# Autodesk Inventor assembly: body assy
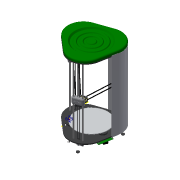
[picture p0: Inventor's stored thumbnail of the model, 180x180]
Saved by Autodesk Inventor 2016 (Build 200138000, 138)
## iProperties
Created: 2016-12-29
Part Number: body assy
Document SubType Name: Assembly
Designer: admin
Author: admin
## Documents named in this file (21)
- C:\Users\Juny\OneDrive - (주)에이팀벤처스\ateam\CL 3D프린터 사업- 설계 이준영\(((( delta 3D printer))))\20. 20190104 D3\1612 D3 3D modeling\body assy.iam
- C:\Users\Juny\OneDrive - (주)에이팀벤처스\ateam\CL 3D프린터 사업- 설계 이준영\(((( delta 3D printer))))\20. 20190104 D3\1612 D3 3D modeling\m3 6 socket_screw.ipt
- C:\Users\Juny\OneDrive - (주)에이팀벤처스\ateam\CL 3D프린터 사업- 설계 이준영\(((( delta 3D printer))))\20. 20190104 D3\1612 D3 3D modeling\m3 8 socket_screw.ipt
- C:\Users\Juny\OneDrive - (주)에이팀벤처스\ateam\CL 3D프린터 사업- 설계 이준영\(((( delta 3D printer))))\20. 20190104 D3\1612 D3 3D modeling\M3 16 BH_tapping_screw.ipt
- C:\Users\Juny\OneDrive - (주)에이팀벤처스\ateam\CL 3D프린터 사업- 설계 이준영\(((( delta 3D printer))))\20. 20190104 D3\1612 D3 3D modeling\m3 30 pcb_support.ipt
- C:\Users\Juny\OneDrive - (주)에이팀벤처스\ateam\CL 3D프린터 사업- 설계 이준영\(((( delta 3D printer))))\20. 20190104 D3\1612 D3 3D modeling\m4 10 Button Head.ipt
- C:\Users\Juny\OneDrive - (주)에이팀벤처스\ateam\CL 3D프린터 사업- 설계 이준영\(((( delta 3D printer))))\20. 20190104 D3\1612 D3 3D modeling\m4 12 Button Head.ipt
- C:\Users\Juny\OneDrive - (주)에이팀벤처스\ateam\CL 3D프린터 사업- 설계 이준영\(((( delta 3D printer))))\20. 20190104 D3\1612 D3 3D modeling\m4 20 Button Head.ipt
- C:\Users\Juny\OneDrive - (주)에이팀벤처스\ateam\CL 3D프린터 사업- 설계 이준영\(((( delta 3D printer))))\20. 20190104 D3\1612 D3 3D modeling\main_board.ipt
- C:\Users\Juny\OneDrive - (주)에이팀벤처스\ateam\CL 3D프린터 사업- 설계 이준영\(((( delta 3D printer))))\20. 20190104 D3\1612 D3 3D modeling\post.ipt
- C:\Users\Juny\OneDrive - (주)에이팀벤처스\ateam\CL 3D프린터 사업- 설계 이준영\(((( delta 3D printer))))\20. 20190104 D3\1612 D3 3D modeling\timing_belt.ipt
- C:\Users\Juny\OneDrive - (주)에이팀벤처스\ateam\CL 3D프린터 사업- 설계 이준영\(((( delta 3D printer))))\20. 20190104 D3\1612 D3 3D modeling\top_cover.ipt
- C:\Users\Juny\OneDrive - (주)에이팀벤처스\ateam\CL 3D프린터 사업- 설계 이준영\(((( delta 3D printer))))\20. 20190104 D3\1612 D3 3D modeling\back_cover.ipt
- C:\Users\Juny\OneDrive - (주)에이팀벤처스\ateam\CL 3D프린터 사업- 설계 이준영\(((( delta 3D printer))))\20. 20190104 D3\1612 D3 3D modeling\bottom cover assy\bottom cover assy.iam
- C:\Users\Juny\OneDrive - (주)에이팀벤처스\ateam\CL 3D프린터 사업- 설계 이준영\(((( delta 3D printer))))\20. 20190104 D3\1612 D3 3D modeling\bottom plate assy\bottom plate assy.iam
- C:\Users\Juny\OneDrive - (주)에이팀벤처스\ateam\CL 3D프린터 사업- 설계 이준영\(((( delta 3D printer))))\20. 20190104 D3\1612 D3 3D modeling\head assy\head assy.iam
- C:\Users\Juny\OneDrive - (주)에이팀벤처스\ateam\CL 3D프린터 사업- 설계 이준영\(((( delta 3D printer))))\20. 20190104 D3\1612 D3 3D modeling\lift block assy\lift block assy.iam
- C:\Users\Juny\OneDrive - (주)에이팀벤처스\ateam\CL 3D프린터 사업- 설계 이준영\(((( delta 3D printer))))\20. 20190104 D3\1612 D3 3D modeling\lod assy\lod assy.iam
- C:\Users\Juny\OneDrive - (주)에이팀벤처스\ateam\CL 3D프린터 사업- 설계 이준영\(((( delta 3D printer))))\20. 20190104 D3\1612 D3 3D modeling\motor assy\motor assy.iam
- C:\Users\Juny\OneDrive - (주)에이팀벤처스\ateam\CL 3D프린터 사업- 설계 이준영\(((( delta 3D printer))))\20. 20190104 D3\1612 D3 3D modeling\oled assy\oled assy.iam
- C:\Users\Juny\OneDrive - (주)에이팀벤처스\ateam\CL 3D프린터 사업- 설계 이준영\(((( delta 3D printer))))\20. 20190104 D3\1612 D3 3D modeling\top plate assy\top plate assy.iam
## Components (64 placed, 20 different names)
1. m3 6 socket_screw:1 — Rotational:39
2. M3 16 BH_tapping_screw:1 — Rotational:18
3. m3 30 pcb_support:1 — Rotational:33
4. m4 10 Button Head:1 — Rotational:25
5. m4 12 Button Head:1 — Rotational:32
6. main_board:1 — Rotational:37, Rotational:38, Rotational:39, Rotational:40, Rotational:41, Rotational:42
7. top_cover:1 — Rotational:23, Rotational:24
8. back_cover:1 — Rotational:21, Rotational:22, Rotational:25, Rotational:26, Rotational:27, Rotational:28, Rotational:29, Rotational:30, Rotational:31, Rotational:32
9. bottom cover assy:1 [sub-assembly] — Rotational:43, Rotational:44
10. bottom plate assy:1 [sub-assembly] — Rotational:3, Rotational:4, Rotational:5, Rotational:6, Rotational:7, Rotational:8, Rotational:21, Rotational:22, Angle:1, Angle:3, Angle:4, Rotational:33, Rotational:34, Rotational:35, Rotational:36, Rotational:43, Rotational:44
11. head assy:1 [sub-assembly] — Tangent:7, Tangent:8, Tangent:9, Tangent:10, Tangent:11, Tangent:12
12. lod assy:1 [sub-assembly] — Tangent:1, Tangent:8
13. oled assy:1 [sub-assembly] — Rotational:5, Rotational:6, Rotational:14, Rotational:15, Rotational:16, Rotational:17
14. top plate assy:1 [sub-assembly] — Rotational:1, Rotational:2, Rotational:11, Rotational:12, Rotational:13, Rotational:18, Rotational:19, Rotational:20, Rotational:23, Rotational:24
15. m3 8 socket_screw:2 — Rotational:14
16. m3 8 socket_screw:3 — Rotational:15
17. m3 8 socket_screw:4 — Rotational:16
18. m3 8 socket_screw:5 — Rotational:17
19. M3 16 BH_tapping_screw:2 — Rotational:19
20. M3 16 BH_tapping_screw:3 — Rotational:20
21. lift block assy:1 [sub-assembly] — Mate:1, Angle:1, Tangent:1, Tangent:2
22. lift block assy:2 [sub-assembly] — Mate:3, Angle:4, Tangent:3, Tangent:4
23. lift block assy:3 [sub-assembly] — Mate:2, Angle:3, Tangent:5, Tangent:6
24. m4 10 Button Head:2 — Rotational:26
25. m4 10 Button Head:3 — Rotational:27
26. m4 10 Button Head:4 — Rotational:28
27. m4 12 Button Head:2 — Rotational:31
28. m4 12 Button Head:3 — Rotational:30
29. m4 12 Button Head:4 — Rotational:29
30. m3 30 pcb_support:2 — Rotational:36
31. m3 30 pcb_support:3 — Rotational:35, Rotational:37
32. m3 30 pcb_support:4 — Rotational:34, Rotational:38
33. m3 6 socket_screw:2 — Rotational:40
34. m3 6 socket_screw:3 — Rotational:41
35. m3 6 socket_screw:4 — Rotational:42
36. lod assy:2 [sub-assembly] — Tangent:2, Tangent:7
37. lod assy:3 [sub-assembly] — Tangent:3, Tangent:11
38. lod assy:4 [sub-assembly] — Tangent:4, Tangent:12
39. lod assy:5 [sub-assembly] — Tangent:5, Tangent:10
40. lod assy:6 [sub-assembly] — Tangent:6, Tangent:9
41. post:2 — Rotational:1, Rotational:3, Mate:2
42. timing_belt:1 — Rotational:13, Cylindrical:1
43. post:1 — Rotational:2, Rotational:4
44. m4 20 Button Head:4 — Rotational:12
45. m4 20 Button Head:3 — Rotational:11
46. m4 20 Button Head:1 — Rotational:9
47. m4 20 Button Head:2 — Rotational:10
48. motor assy:1 [sub-assembly] — Rotational:7, Rotational:8, Rotational:9, Rotational:10, Cylindrical:1
49. post:3 — Mate:3
50. timing_belt:2
51. post:4
52. m4 20 Button Head:5
53. m4 20 Button Head:6
54. m4 20 Button Head:7
55. m4 20 Button Head:8
56. motor assy:2 [sub-assembly]
57. post:5
58. timing_belt:3
59. post:6 — Mate:1
60. m4 20 Button Head:9
61. m4 20 Button Head:10
62. m4 20 Button Head:11
63. m4 20 Button Head:12
64. motor assy:3 [sub-assembly]
## Component patterns: (3 elements, first: post:2 + timing_belt:1 + post:1 + m4 20 Button Head:4 + m4 20 Button Head:3 + m4 20 Button Head:1 + m4 20 Button Head:2 + motor assy:1)
## Relationships (63: RevoluteJoint 44, Tangent 12, Mate 3, Angle 3, CylindricalJoint 1)
- Rotational:1 [RevoluteJoint]: top plate assy:1 ↔ post:2
- Rotational:2 [RevoluteJoint]: top plate assy:1 ↔ post:1
- Rotational:3 [RevoluteJoint]: bottom plate assy:1 ↔ post:2
- Rotational:4 [RevoluteJoint]: bottom plate assy:1 ↔ post:1
- Rotational:5 [RevoluteJoint]: bottom plate assy:1 ↔ oled assy:1
- Rotational:6 [RevoluteJoint]: bottom plate assy:1 ↔ oled assy:1
- Rotational:7 [RevoluteJoint]: bottom plate assy:1 ↔ motor assy:1
- Rotational:8 [RevoluteJoint]: bottom plate assy:1 ↔ motor assy:1
- Rotational:9 [RevoluteJoint]: m4 20 Button Head:1 ↔ motor assy:1
- Rotational:10 [RevoluteJoint]: m4 20 Button Head:2 ↔ motor assy:1
- Rotational:11 [RevoluteJoint]: top plate assy:1 ↔ m4 20 Button Head:3
- Rotational:12 [RevoluteJoint]: top plate assy:1 ↔ m4 20 Button Head:4
- Rotational:13 [RevoluteJoint]: top plate assy:1 ↔ timing_belt:1
- Cylindrical:1: timing_belt:1 ↔ motor assy:1
- Rotational:14 [RevoluteJoint]: oled assy:1 ↔ m3 8 socket_screw:2
- Rotational:15 [RevoluteJoint]: oled assy:1 ↔ m3 8 socket_screw:3
- Rotational:16 [RevoluteJoint]: oled assy:1 ↔ m3 8 socket_screw:4
- Rotational:17 [RevoluteJoint]: oled assy:1 ↔ m3 8 socket_screw:5
- Rotational:18 [RevoluteJoint]: M3 16 BH_tapping_screw:1 ↔ top plate assy:1
- Rotational:19 [RevoluteJoint]: top plate assy:1 ↔ M3 16 BH_tapping_screw:2
- Rotational:20 [RevoluteJoint]: top plate assy:1 ↔ M3 16 BH_tapping_screw:3
- Rotational:21 [RevoluteJoint]: back_cover:1 ↔ bottom plate assy:1
- Rotational:22 [RevoluteJoint]: back_cover:1 ↔ bottom plate assy:1
- Rotational:23 [RevoluteJoint]: top_cover:1 ↔ top plate assy:1
- Rotational:24 [RevoluteJoint]: top_cover:1 ↔ top plate assy:1
- Mate:1: lift block assy:1 ↔ post:6
- Angle:1 (0 deg): bottom plate assy:1 ↔ lift block assy:1
- Mate:2: lift block assy:3 ↔ post:2
- Angle:3 (0 deg): bottom plate assy:1 ↔ lift block assy:3
- Mate:3: lift block assy:2 ↔ post:3
- Angle:4 (0 deg): bottom plate assy:1 ↔ lift block assy:2
- Rotational:25 [RevoluteJoint]: m4 10 Button Head:1 ↔ back_cover:1
- Rotational:26 [RevoluteJoint]: back_cover:1 ↔ m4 10 Button Head:2
- Rotational:27 [RevoluteJoint]: back_cover:1 ↔ m4 10 Button Head:3
- Rotational:28 [RevoluteJoint]: back_cover:1 ↔ m4 10 Button Head:4
- Rotational:29 [RevoluteJoint]: back_cover:1 ↔ m4 12 Button Head:4
- Rotational:30 [RevoluteJoint]: back_cover:1 ↔ m4 12 Button Head:3
- Rotational:31 [RevoluteJoint]: back_cover:1 ↔ m4 12 Button Head:2
- Rotational:32 [RevoluteJoint]: m4 12 Button Head:1 ↔ back_cover:1
- Rotational:33 [RevoluteJoint]: m3 30 pcb_support:1 ↔ bottom plate assy:1
- Rotational:34 [RevoluteJoint]: bottom plate assy:1 ↔ m3 30 pcb_support:4
- Rotational:35 [RevoluteJoint]: bottom plate assy:1 ↔ m3 30 pcb_support:3
- Rotational:36 [RevoluteJoint]: bottom plate assy:1 ↔ m3 30 pcb_support:2
- Rotational:37 [RevoluteJoint]: main_board:1 ↔ m3 30 pcb_support:3
- Rotational:38 [RevoluteJoint]: main_board:1 ↔ m3 30 pcb_support:4
- Rotational:39 [RevoluteJoint]: m3 6 socket_screw:1 ↔ main_board:1
- Rotational:40 [RevoluteJoint]: main_board:1 ↔ m3 6 socket_screw:2
- Rotational:41 [RevoluteJoint]: main_board:1 ↔ m3 6 socket_screw:3
- Rotational:42 [RevoluteJoint]: main_board:1 ↔ m3 6 socket_screw:4
- Rotational:43 [RevoluteJoint]: bottom cover assy:1 ↔ bottom plate assy:1
- Rotational:44 [RevoluteJoint]: bottom cover assy:1 ↔ bottom plate assy:1
- Tangent:1: lod assy:1 ↔ lift block assy:1
- Tangent:2: lift block assy:1 ↔ lod assy:2
- Tangent:3: lift block assy:2 ↔ lod assy:3
- Tangent:4: lift block assy:2 ↔ lod assy:4
- Tangent:5: lift block assy:3 ↔ lod assy:5
- Tangent:6: lift block assy:3 ↔ lod assy:6
- Tangent:7: head assy:1 ↔ lod assy:2
- Tangent:8: head assy:1 ↔ lod assy:1
- Tangent:9: head assy:1 ↔ lod assy:6
- Tangent:10: head assy:1 ↔ lod assy:5
- Tangent:11: head assy:1 ↔ lod assy:3
- Tangent:12: head assy:1 ↔ lod assy:4
